# Autodesk Inventor assembly: Zespół2
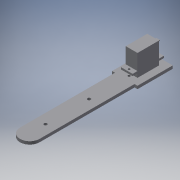
[picture p0: Inventor's stored thumbnail of the model, 180x180]
Saved by Autodesk Inventor 2017 (Build 210142000, 142)
## iProperties
Part Number: Zespół2
Material: Ogólny
Document SubType Name: Assembly
Designer: Damian
Author: Damian
## Documents named in this file (3)
- C:\Users\Damian\Documents\Inventor\Nowe\2.0\Zespół2.iam
- C:\Users\Damian\Documents\Inventor\Nowe\towerpro.ipt
- C:\Users\Damian\Documents\Inventor\Nowe\2.0\Część2.ipt
## Components (2 placed, 2 different names)
1. towerpro:1 — Wstaw:1, Zestawiający:1
2. Część2:1 — Wstaw:1, Zestawiający:1
## Relationships (2: Insert 1, Mate 1)
- Wstaw:1 [Insert] (-4 mm): towerpro:1 ↔ Część2:1
- Zestawiający:1 [Mate] (6 mm): towerpro:1 ↔ Część2:1
